# Autodesk Inventor assembly: Assembly
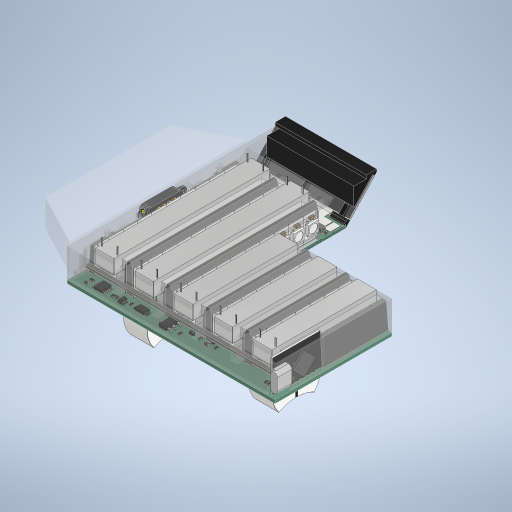
[picture p0: Inventor's stored thumbnail of the model, 512x512]
Saved by Autodesk Inventor 2023 (Build 270158000, 158)
## iProperties
Created: 2024-03-19
Part Number: Assembly
Document SubType Name: Assembly
Designer: noname
Author: noname
## iProperties of the stored document SOT-23-6.iam
Created: 2024-03-26
Part Number: SOT-23-6
Document SubType Name: Assembly
Designer: noname
Author: noname
## iProperties of the stored document D_SOD_323.ipt
Created: 2024-03-26
Part Number: D_SOD_323
Material: Generic
Document SubType Name: Modeling
Designer: noname
Density: 1 g/cm^3
Appearance: Default
Author: noname
## iProperties of the stored document AudMix_PCB.ipt
Created: 2024-03-26
Part Number: AudMix_PCB
Material: Generic
Document SubType Name: Modeling
Designer: noname
Density: 1 g/cm^3
Appearance: Default
Author: noname
## iProperties of the stored document HSOP-8-1EP_3.9x4.9mm_P1.27mm_EP2.41x3.1mm.iam
Created: 2024-03-26
Part Number: HSOP-8-1EP_3.9x4.9mm_P1.27mm_EP2.41x3.1mm
Document SubType Name: Assembly
Designer: noname
Author: noname
## iProperties of the stored document SOT-223.iam
Created: 2024-03-26
Part Number: SOT-223
Document SubType Name: Assembly
Designer: noname
Author: noname
## iProperties of the stored document TopBoardPCB.iam
Company: Kicad
Created: 2024-03-26
Part Number: TopBoardPCB 1
Description: KiCad electronic assembly
Document SubType Name: Assembly
Designer: noname
Authority: Unknown
Sending System: KiCad to STEP converter
Preprocessor: Open CASCADE STEP processor 7.7
Title: TopBoardPCB.step
Author: Pcbnew
## iProperties of the stored document HSOP_8_1EP_39x49mm_P127mm_EP241x31mm.ipt
Created: 2024-03-26
Part Number: HSOP_8_1EP_39x49mm_P127mm_EP241x31mm
Material: Generic
Document SubType Name: Modeling
Designer: noname
Density: 1 g/cm^3
Appearance: Default
Author: noname
## iProperties of the stored document SOT_23_6.ipt
Created: 2024-03-26
Part Number: SOT_23_6
Material: Generic
Document SubType Name: Modeling
Designer: noname
Density: 1 g/cm^3
Appearance: Default
Author: noname
## iProperties of the stored document TSSOP-8_4.4x3mm_P0.65mm.iam
Created: 2024-03-26
Part Number: TSSOP-8_4.4x3mm_P0.65mm
Document SubType Name: Assembly
Designer: noname
Author: noname
## iProperties of the stored document TSSOP_8_44x3mm_P065mm.ipt
Created: 2024-03-26
Part Number: TSSOP_8_44x3mm_P065mm
Material: Generic
Document SubType Name: Modeling
Designer: noname
Density: 1 g/cm^3
Appearance: Default
Author: noname
## iProperties of the stored document SOT_223.ipt
Created: 2024-03-26
Part Number: SOT_223
Material: Generic
Document SubType Name: Modeling
Designer: noname
Density: 1 g/cm^3
Appearance: Default
Author: noname
## iProperties of the stored document D_SOD-323.iam
Created: 2024-03-26
Part Number: D_SOD-323
Document SubType Name: Assembly
Designer: noname
Author: noname
## iProperties of the stored document LED_WS2812B_PLCC4_5.0x5.0mm_P3.2mm.iam
Created: 2024-03-26
Part Number: LED_WS2812B_PLCC4_5.0x5.0mm_P3.2mm
Document SubType Name: Assembly
Designer: noname
Author: noname
## iProperties of the stored document C_0603_1608Metric.ipt
Created: 2024-03-26
Part Number: C_0603_1608Metric
Material: Generic
Document SubType Name: Modeling
Designer: noname
Density: 1 g/cm^3
Appearance: Default
Author: noname
## iProperties of the stored document R_0603_1608Metric.iam
Created: 2024-03-26
Part Number: R_0603_1608Metric
Document SubType Name: Assembly
Designer: noname
Author: noname
## iProperties of the stored document C_0603_1608Metric.iam
Created: 2024-03-26
Part Number: C_0603_1608Metric
Document SubType Name: Assembly
Designer: noname
Author: noname
## iProperties of the stored document LED_WS2812B_PLCC4_50x50mm_P32mm.ipt
Created: 2024-03-26
Part Number: LED_WS2812B_PLCC4_50x50mm_P32mm
Material: Generic
Document SubType Name: Modeling
Designer: noname
Density: 1 g/cm^3
Appearance: Default
Author: noname
## iProperties of the stored document R_0603_1608Metric.ipt
Created: 2024-03-26
Part Number: R_0603_1608Metric
Material: Generic
Document SubType Name: Modeling
Designer: noname
Density: 1 g/cm^3
Appearance: Default
Author: noname
## Documents named in this file (27)
- C:\Users\noname\Documents\GitHub\AudMix\3dModels\Assembly.iam
- C:\Users\noname\Documents\GitHub\AudMix\3dModels\0_42_oled.ipt
- C:\Users\noname\Documents\GitHub\AudMix\3dModels\rp2040.ipt
- C:\Users\noname\Documents\GitHub\AudMix\3dModels\Front.ipt
- C:\Users\noname\Documents\GitHub\AudMix\3dModels\Case.ipt
- C:\Users\noname\Documents\GitHub\AudMix\3dModels\Connector2.ipt
- **C:\Users\noname\Documents\GitHub\AudMix\3dModels\Assembly.iam*LocalDocs*xAaaaaoaaAaaaaaaaAaaaquxf1b*TopBoardPCB.iam
- C:\Users\noname\Documents\GitHub\AudMix\3dModels\ButtonPanel.ipt
- C:\Users\noname\Documents\GitHub\AudMix\3dModels\Sliders block.iam
- **C:\Users\noname\Documents\GitHub\AudMix\3dModels\Assembly.iam*LocalDocs*xAaaaarbaAaaaaaaaAaaaq5teJd*SOT-23-6.iam
- **C:\Users\noname\Documents\GitHub\AudMix\3dModels\Assembly.iam*LocalDocs*xAaaaaqbaAaaaaaaaAaaaagffJd*SOT_23_6.ipt
- **C:\Users\noname\Documents\GitHub\AudMix\3dModels\Assembly.iam*LocalDocs*xAaaaaiaaAaaaaaaaAaaaa0jcAh*D_SOD_323.ipt
- **C:\Users\noname\Documents\GitHub\AudMix\3dModels\Assembly.iam*LocalDocs*xAaaaabbaAaaaaaaaAaaaqenhUe*AudMix_PCB.ipt
- **C:\Users\noname\Documents\GitHub\AudMix\3dModels\Assembly.iam*LocalDocs*xAaaaa2caAaaaaaaaAaaaay4eEh*HSOP-8-1EP_3.9x4.9mm_P1.27mm_EP2.41x3.1mm.iam
- **C:\Users\noname\Documents\GitHub\AudMix\3dModels\Assembly.iam*LocalDocs*xAaaaakbaAaaaaaaaAaaaazje4g*HSOP_8_1EP_39x49mm_P127mm_EP241x31mm.ipt
- **C:\Users\noname\Documents\GitHub\AudMix\3dModels\Assembly.iam*LocalDocs*xAaaaahbaAaaaaaaaAaaaqjiiQg*SOT-223.iam
- **C:\Users\noname\Documents\GitHub\AudMix\3dModels\Assembly.iam*LocalDocs*xAaaaasbaAaaaaaaaAaaaqcrn4a*SOT_223.ipt
- **C:\Users\noname\Documents\GitHub\AudMix\3dModels\Assembly.iam*LocalDocs*xAaaaqkaaAaaaaaaaAaaaqzje5d*LED_WS2812B_PLCC4_5.0x5.0mm_P3.2mm.iam
- **C:\Users\noname\Documents\GitHub\AudMix\3dModels\Assembly.iam*LocalDocs*xAaaaqlbaAaaaaaaaAaaaqtflXc*C_0603_1608Metric.iam
- **C:\Users\noname\Documents\GitHub\AudMix\3dModels\Assembly.iam*LocalDocs*xAaaaqocaAaaaaaaaAaaaat0d4h*R_0603_1608Metric.iam
- **C:\Users\noname\Documents\GitHub\AudMix\3dModels\Assembly.iam*LocalDocs*xAaaaaudaAaaaaaaaAaaaq33oOg*D_SOD-323.iam
- **C:\Users\noname\Documents\GitHub\AudMix\3dModels\Assembly.iam*LocalDocs*xAaaaq5caAaaaaaaaAaaaqejqYa*TSSOP-8_4.4x3mm_P0.65mm.iam
- **C:\Users\noname\Documents\GitHub\AudMix\3dModels\Assembly.iam*LocalDocs*xAaaaascaAaaaaaaaAaaaavk2Ge*TSSOP_8_44x3mm_P065mm.ipt
- **C:\Users\noname\Documents\GitHub\AudMix\3dModels\Assembly.iam*LocalDocs*xAaaaqpcaAaaaaaaaAaaaqouu3a*LED_WS2812B_PLCC4_50x50mm_P32mm.ipt
- **C:\Users\noname\Documents\GitHub\AudMix\3dModels\Assembly.iam*LocalDocs*xAaaaqhaaAaaaaaaaAaaaqepwHb*C_0603_1608Metric.ipt
- **C:\Users\noname\Documents\GitHub\AudMix\3dModels\Assembly.iam*LocalDocs*xAaaaqsdaAaaaaaaaAaaaqkis4e*R_0603_1608Metric.ipt
- C:\Users\noname\Documents\GitHub\AudMix\3dModels\TopBoardPCB.step
## Components (12 placed, 8 different names)
1. rp2040:1 — Flush:39, Mate:37, Mate:38
2. Front:1 — Mate:32, Mate:33, Flush:38, Mate:34, Mate:35, Mate:36
3. Case:1 — Mate:26, Flush:36, Flush:37, Mate:27, Rotational:1, Mate:28
4. TopBoardPCB:1 [sub-assembly] — Mate:26, Flush:36, Flush:37, Mate:29, Mate:30, Mate:31, Mate:32, Mate:33, Flush:38, Flush:39, Mate:37, Mate:38
5. Connector2:2 — Mate:27, Rotational:1, Angle:1
6. ButtonPanel:1 — Mate:28
7. Sliders block:1 [sub-assembly] — Mate:29, Mate:30, Mate:31, Angle:1
8. 0_42_oled:5 — Mate:34, Mate:35, Mate:36
9. 0_42_oled:6
10. 0_42_oled:7
11. 0_42_oled:8
12. 0_42_oled:9
## Component patterns: (5 elements, first: 0_42_oled:5)
## Relationships (19: Mate 13, Flush 4, RevoluteJoint 1, Angle 1)
- Mate:26: Case:1 ↔ TopBoardPCB:1
- Flush:36: Case:1 ↔ TopBoardPCB:1
- Flush:37: Case:1 ↔ TopBoardPCB:1
- Mate:27: Case:1 ↔ Connector2:2
- Rotational:1 [RevoluteJoint]: Case:1 ↔ Connector2:2
- Mate:28: Case:1 ↔ ButtonPanel:1
- Mate:29: TopBoardPCB:1 ↔ Sliders block:1
- Mate:30: TopBoardPCB:1 ↔ Sliders block:1
- Mate:31: TopBoardPCB:1 ↔ Sliders block:1
- Angle:1 (180 deg): Connector2:2 ↔ Sliders block:1
- Mate:32: Front:1 ↔ TopBoardPCB:1
- Mate:33: Front:1 ↔ TopBoardPCB:1
- Flush:38: Front:1 ↔ TopBoardPCB:1
- Mate:34 (0.5 mm): Front:1 ↔ 0_42_oled:5
- Mate:35 (0.1 mm): Front:1 ↔ 0_42_oled:5
- Mate:36 (0.3 mm): Front:1 ↔ 0_42_oled:5
- Flush:39 (-1 mm): rp2040:1 ↔ TopBoardPCB:1
- Mate:37 (0.05 mm): rp2040:1 ↔ TopBoardPCB:1
- Mate:38: rp2040:1 ↔ TopBoardPCB:1
